# Autodesk Inventor assembly: PlateRailClamp48in
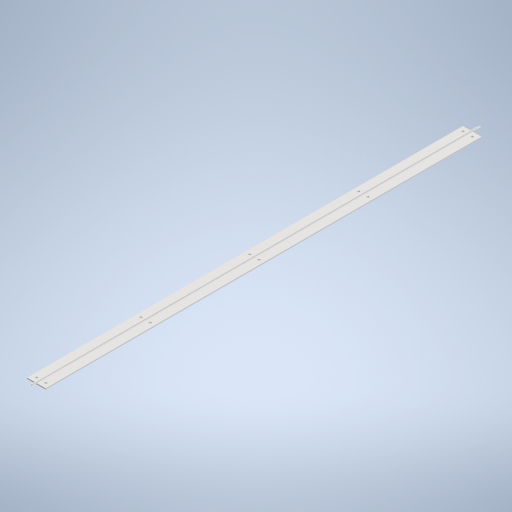
[picture p0: Inventor's stored thumbnail of the model, 512x512]
Saved by Autodesk Inventor 2023 (Build 270158030, 158C)
## iProperties
Created: 2023-02-14
Part Number: PlateRailClamp48in
Document SubType Name: Assembly
Designer: jeremyy
Author: jeremyy
## Documents named in this file (4)
- \\andrew.ad.cmu.edu\users\users1\jeremyy\Documents\Inventor\CMU Bridge\New folder\PlateRailClamp48in.iam
- \\andrew.ad.cmu.edu\users\users1\jeremyy\Documents\Inventor\CMU Bridge\New folder\Plate2inx47in.ipt
- \\andrew.ad.cmu.edu\users\users1\jeremyy\Documents\Inventor\CMU Bridge\New folder\Rail48in.ipt
- \\andrew.ad.cmu.edu\users\users1\jeremyy\Documents\Inventor\CMU Bridge\New folder\RailClamp.ipt
## Components (3 placed, 3 different names)
1. Plate2inx47in:1 — Mate:1, Flush:1, Flush:2, Mate:4
2. Rail48in:1 — Mate:1, Flush:1, Flush:2, Mate:2, Mate:3
3. RailClamp:1 — Mate:2, Mate:3, Mate:4
## Relationships (6: Mate 4, Flush 2)
- Mate:1: Plate2inx47in:1 ↔ Rail48in:1
- Flush:1 (-12.7 mm): Plate2inx47in:1 ↔ Rail48in:1
- Flush:2 (23.5458 mm): Plate2inx47in:1 ↔ Rail48in:1
- Mate:2: Rail48in:1 ↔ RailClamp:1
- Mate:3: Rail48in:1 ↔ RailClamp:1
- Mate:4 (3.175 mm): Plate2inx47in:1 ↔ RailClamp:1
